# Autodesk Inventor assembly: Base_AX12
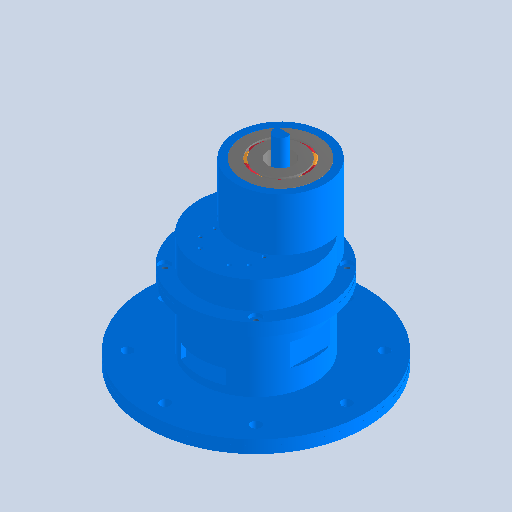
[picture p0: Inventor's stored thumbnail of the model, 512x512]
Saved by Autodesk Inventor 2024 (Build 280153000, 153)
## iProperties
Created: 2022-06-07
Part Number: Base_AX12
Document SubType Name: Assembly
Designer: Alcatraz
Author: Alcatraz
## Documents named in this file (7)
- C:\Users\Alcatraz\Desktop\TESIS-actual\Lista_Piezas_MovPlano_21Junio\Lista_Piezas\Base-AX12\Base_AX12.iam
- C:\Users\Alcatraz\Desktop\TESIS-actual\Lista_Piezas\Rodamiento_Giro_V7\Rodamiento_Giro_V7.iam
- C:\Users\Alcatraz\Desktop\TESIS-actual\Lista_Piezas_MovPlano_21Junio\Lista_Piezas\Base-AX12\B-01.ipt
- C:\Users\Alcatraz\Desktop\TESIS-actual\Lista_Piezas_MovPlano_21Junio\Lista_Piezas\Base-AX12\B-02.ipt
- C:\Users\Alcatraz\Desktop\TESIS-actual\Lista_Piezas_MovPlano_21Junio\Lista_Piezas\Base-AX12\B-03.ipt
- C:\Users\Alcatraz\Desktop\TESIS-actual\Lista_Piezas\Bridas\BM-AX12.ipt
- C:\Users\Alcatraz\Desktop\TESIS-actual\Lista_Piezas\AX-12A,18A,12W,MX-12W(stp)\AX-12A.iam
## Components (7 placed, 6 different names)
1. Rodamiento_Giro_V7:1 [sub-assembly] — Coincidencia:4, Coincidencia:5, Coincidencia:12
2. Rodamiento_Giro_V7:2 [sub-assembly] — Coincidencia:4, Coincidencia:5, Coincidencia:13
3. B-01:1 — Coincidencia:14, Coincidencia:15, Coincidencia:16
4. B-02:1 — Coincidencia:1, Coincidencia:2, Coincidencia:3, Coincidencia:6, Coincidencia:7, Coincidencia:8, Coincidencia:14, Coincidencia:15, Coincidencia:16
5. B-03:1 — Coincidencia:6, Coincidencia:7, Coincidencia:8, Coincidencia:13
6. BM-AX12:1 — Coincidencia:9, Coincidencia:10, Coincidencia:11, Coincidencia:12
7. AX-12A:1 [sub-assembly] — Coincidencia:1, Coincidencia:2, Coincidencia:3, Coincidencia:9, Coincidencia:10, Coincidencia:11
## Relationships (16: Mate 16)
- Coincidencia:1 [Mate]: B-02:1 ↔ AX-12A:1
- Coincidencia:2 [Mate]: B-02:1 ↔ AX-12A:1
- Coincidencia:3 [Mate]: B-02:1 ↔ AX-12A:1
- Coincidencia:4 [Mate]: Rodamiento_Giro_V7:1 ↔ Rodamiento_Giro_V7:2
- Coincidencia:5 [Mate]: Rodamiento_Giro_V7:1 ↔ Rodamiento_Giro_V7:2
- Coincidencia:6 [Mate]: B-02:1 ↔ B-03:1
- Coincidencia:7 [Mate]: B-02:1 ↔ B-03:1
- Coincidencia:8 [Mate]: B-02:1 ↔ B-03:1
- Coincidencia:9 [Mate]: BM-AX12:1 ↔ AX-12A:1
- Coincidencia:10 [Mate]: BM-AX12:1 ↔ AX-12A:1
- Coincidencia:11 [Mate]: BM-AX12:1 ↔ AX-12A:1
- Coincidencia:12 [Mate]: Rodamiento_Giro_V7:1 ↔ BM-AX12:1
- Coincidencia:13 [Mate]: Rodamiento_Giro_V7:2 ↔ B-03:1
- Coincidencia:14 [Mate]: B-01:1 ↔ B-02:1
- Coincidencia:15 [Mate]: B-01:1 ↔ B-02:1
- Coincidencia:16 [Mate]: B-01:1 ↔ B-02:1
